# Autodesk Inventor assembly: Assembly1
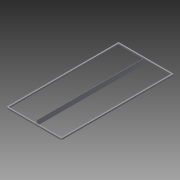
[picture p0: Inventor's stored thumbnail of the model, 180x180]
Saved by Autodesk Inventor 2015 SP1 (Build 190203100, 203)
## iProperties
Created: 2015-03-28
Part Number: Assembly1
Document SubType Name: Assembly
Designer: Cyril
Author: Cyril
## Documents named in this file (6)
- C:\Users\Cyril\Documents\OSE FR\Concentrateur solaire\Assembly1.iam
- C:\Users\Cyril\Documents\OSE FR\Concentrateur solaire\Part1.ipt
- C:\Users\Cyril\Documents\OSE FR\Concentrateur solaire\Part2.ipt
- C:\Users\Cyril\Documents\OSE FR\Concentrateur solaire\Mirroir.ipt
- C:\Users\Cyril\Documents\OSE FR\Concentrateur solaire\Part3.ipt
- C:\Users\Cyril\Documents\OSE FR\Concentrateur solaire\Part4.ipt
## Components (7 placed, 5 different names)
1. Part1:1 — Flush:5, Mate:2, Flush:6, Mate:3, Flush:7, Flush:8
2. Part1:2 — Mate:1, Flush:3, Flush:4
3. Part2:1 — Mate:3, Flush:7, Flush:8
4. Part2:2 — Mate:1, Flush:3, Flush:4, Flush:5, Mate:2, Flush:6, Mate:5, Flush:9
5. Mirroir:1 — Mate:6, Mate:7, Mate:8
6. Part3:1 — Insert:1, Mate:6, Mate:7, Mate:8
7. Part4:1 — Mate:5, Flush:9, Insert:1
## Relationships (15: Mate 7, Flush 7, Insert 1)
- Mate:1: Part1:2 ↔ Part2:2
- Flush:3: Part1:2 ↔ Part2:2
- Flush:4: Part1:2 ↔ Part2:2
- Flush:5: Part1:1 ↔ Part2:2
- Mate:2: Part1:1 ↔ Part2:2
- Flush:6: Part1:1 ↔ Part2:2
- Mate:3: Part1:1 ↔ Part2:1
- Flush:7: Part1:1 ↔ Part2:1
- Flush:8: Part1:1 ↔ Part2:1
- Mate:5: Part2:2 ↔ Part4:1
- Flush:9: Part2:2 ↔ Part4:1
- Insert:1: Part3:1 ↔ Part4:1
- Mate:6: Mirroir:1 ↔ Part3:1
- Mate:7 (15 mm): Mirroir:1 ↔ Part3:1
- Mate:8: Mirroir:1 ↔ Part3:1
